# Autodesk Inventor assembly: fan with wheel-01
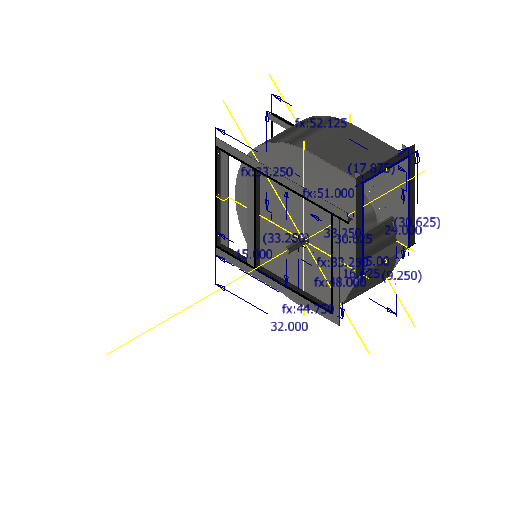
[picture p0: Inventor's stored thumbnail of the model, 512x512]
Saved by Autodesk Inventor 2022 (Build 260148000, 148)
## iProperties
Created: 2007-05-11
Part Number: fan with wheel-01
Document SubType Name: Assembly
Designer: LionelF
Mass: 141500 g
Surface Area: 161564 cm^2
Volume: 28987.6 cm^3
Density: 4.88141 g/cm^3
Author: LionelF
## Documents named in this file (10)
- D:\Autodesk Inventor 2021 Advanced Assembly Modeling Practice Files\Blower\fan with wheel.iam
- D:\Autodesk Inventor 2021 Advanced Assembly Modeling Practice Files\Blower\FAN CONSTRAINED.iam
- D:\Autodesk Inventor 2021 Advanced Assembly Modeling Practice Files\Blower\cover plate.ipt
- D:\Autodesk Inventor 2021 Advanced Assembly Modeling Practice Files\Blower\wheel.ipt
- D:\Autodesk Inventor 2021 Advanced Assembly Modeling Practice Files\Blower\inlet cone.ipt
- D:\Autodesk Inventor 2021 Advanced Assembly Modeling Practice Files\Blower\Inlet Stiffening.iam
- D:\Autodesk Inventor 2021 Advanced Assembly Modeling Practice Files\Blower\Shaftside Stiffening.iam
- D:\Autodesk Inventor 2021 Advanced Assembly Modeling Practice Files\Blower\Coneside Stiffening, Cornered.iam
- D:\Autodesk Inventor 2021 Advanced Assembly Modeling Practice Files\Blower\shaft_blower.ipt
- D:\Autodesk Inventor 2021 Advanced Assembly Modeling Practice Files\Blower\angle test.xls
## Components (8 placed, 8 different names)
1. FAN CONSTRAINED:1 [sub-assembly] — Mate:4, Mate:5, Mate:6, Mate:7, Mate:10, Mate:12, Mate:13, Flush:1, Mate:17, Mate:18
2. cover plate:1 — Mate:5, Mate:6, Mate:7, Mate:8, Mate:9
3. wheel:1 — Mate:1, Mate:2, Mate:3, Mate:4, Mate:11
4. shaft_blower:1 — Mate:1, Mate:2, Mate:3
5. inlet cone:1 — Mate:8, Mate:9, Mate:10, Mate:11, Mate:20
6. Inlet Stiffening:1 [sub-assembly] — Mate:12, Mate:13, Flush:1, Angle:4
7. Shaftside Stiffening:1 [sub-assembly] — Mate:17, Mate:19, Angle:3, Mate:20
8. Coneside Stiffening, Cornered:1 [sub-assembly] — Mate:18, Mate:19, Angle:3, Angle:4
## Relationships (20: Mate 17, Angle 2, Flush 1)
- Mate:1: wheel:1 ↔ shaft_blower:1
- Mate:2: wheel:1 ↔ shaft_blower:1
- Mate:3: wheel:1 ↔ shaft_blower:1
- Mate:4: FAN CONSTRAINED:1 ↔ wheel:1
- Mate:5: FAN CONSTRAINED:1 ↔ cover plate:1
- Mate:6: FAN CONSTRAINED:1 ↔ cover plate:1
- Mate:7: FAN CONSTRAINED:1 ↔ cover plate:1
- Mate:8: cover plate:1 ↔ inlet cone:1
- Mate:9: cover plate:1 ↔ inlet cone:1
- Mate:10: FAN CONSTRAINED:1 ↔ inlet cone:1
- Mate:11 (-6.35 mm): wheel:1 ↔ inlet cone:1
- Mate:12: FAN CONSTRAINED:1 ↔ Inlet Stiffening:1
- Mate:13: FAN CONSTRAINED:1 ↔ Inlet Stiffening:1
- Flush:1: FAN CONSTRAINED:1 ↔ Inlet Stiffening:1
- Mate:17: FAN CONSTRAINED:1 ↔ Shaftside Stiffening:1
- Mate:18: FAN CONSTRAINED:1 ↔ Coneside Stiffening, Cornered:1
- Mate:19: Shaftside Stiffening:1 ↔ Coneside Stiffening, Cornered:1
- Angle:3 (0 deg): Shaftside Stiffening:1 ↔ Coneside Stiffening, Cornered:1
- Mate:20: inlet cone:1 ↔ Shaftside Stiffening:1
- Angle:4 (0 deg): Inlet Stiffening:1 ↔ Coneside Stiffening, Cornered:1
## Named parameters: Discharge_Angle = 0 deg
